# Autodesk Inventor assembly: piston-4in-V03
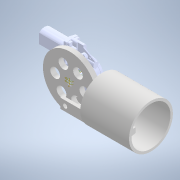
[picture p0: Inventor's stored thumbnail of the model, 180x180]
Saved by Autodesk Inventor 2020.2 (Build 242310000, 310)
## iProperties
Created: 2020-01-21
Part Number: piston-4in-V03
Document SubType Name: Assembly
Designer: robst
Author: robst
## Documents named in this file (6)
- C:\git\CAD-Development\robSteele\2020BallTriggerMechanism\piston-4in-V03.iam
- C:\git\CAD-Development\robSteele\2020BallTriggerMechanism\am-2373 Snow Blower Motor Mount.ipt
- C:\git\CAD-Development\robSteele\2020BallTriggerMechanism\am-2235a Snow Blower Motor With Hex Shaft.iam
- C:\git\CAD-Development\robSteele\2020BallTriggerMechanism\driveForPiston.ipt
- C:\git\CAD-Development\robSteele\2020BallTriggerMechanism\connectiingRodV03.ipt
- C:\git\CAD-Development\robSteele\2020BallTriggerMechanism\cylinder.ipt
## Components (5 placed, 5 different names)
1. am-2373 Snow Blower Motor Mount:1 — Insert:1, Insert:2
2. am-2235a Snow Blower Motor With Hex Shaft:1 [sub-assembly] — Insert:1, Insert:2, Insert:3
3. driveForPiston:1 — Insert:3, Insert:4
4. connectiingRodV03:1 — Insert:4
5. cylinder:1
## Relationships (4: Insert 4)
- Insert:1: am-2373 Snow Blower Motor Mount:1 ↔ am-2235a Snow Blower Motor With Hex Shaft:1
- Insert:2: am-2373 Snow Blower Motor Mount:1 ↔ am-2235a Snow Blower Motor With Hex Shaft:1
- Insert:3: am-2235a Snow Blower Motor With Hex Shaft:1 ↔ driveForPiston:1
- Insert:4: driveForPiston:1 ↔ connectiingRodV03:1
